# Autodesk Inventor assembly: dxdyrrdtr
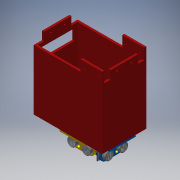
[picture p0: Inventor's stored thumbnail of the model, 180x180]
Saved by Autodesk Inventor 2017 (Build 210142000, 142)
## iProperties
Created: 2017-12-22
Part Number: dxdyrrdtr
Document SubType Name: Assembly
Designer: Dharsan
Author: Dharsan
## Documents named in this file (4)
- C:\Users\Dharsan\Desktop\Dharsan Innovation Files\Cart Model Inventor\Cart Assembly Full.iam
- C:\Users\Dharsan\Desktop\Dharsan Innovation Files\Cart Model Inventor\Cart Body.ipt
- C:\Users\Dharsan\Desktop\Dharsan Innovation Files\Cart Model Inventor\Sensor Hoder and Sensor Assembly.iam
- C:\Users\Dharsan\Desktop\Dharsan Innovation Files\Cart Model Inventor\AS 1427 - M3 x 8(5) II screw.ipt
## Components (7 placed, 3 different names)
1. Cart Body:1 — Mate:8, Mate:9, Mate:10, Mate:11, Mate:12
2. Sensor Hoder and Sensor Assembly:4 [sub-assembly] — Mate:8, Mate:10, Mate:13, Mate:14, Mate:17, Mate:18
3. Sensor Hoder and Sensor Assembly:5 [sub-assembly] — Mate:9, Mate:11, Mate:12, Mate:15, Mate:16, Mate:19, Mate:20
4. AS 1427 - M3 x 8(5) II screw:1 — Mate:19, Mate:20
5. AS 1427 - M3 x 8(5) II screw:2 — Mate:17, Mate:18
6. AS 1427 - M3 x 8(5) II screw:3 — Mate:15, Mate:16
7. AS 1427 - M3 x 8(5) II screw:6 — Mate:13, Mate:14
## Relationships (13: Mate 13)
- Mate:8: Cart Body:1 ↔ Sensor Hoder and Sensor Assembly:4
- Mate:9: Cart Body:1 ↔ Sensor Hoder and Sensor Assembly:5
- Mate:10: Cart Body:1 ↔ Sensor Hoder and Sensor Assembly:4
- Mate:11: Cart Body:1 ↔ Sensor Hoder and Sensor Assembly:5
- Mate:12 (30 mm): Cart Body:1 ↔ Sensor Hoder and Sensor Assembly:5
- Mate:13: Sensor Hoder and Sensor Assembly:4 ↔ AS 1427 - M3 x 8(5) II screw:6
- Mate:14: Sensor Hoder and Sensor Assembly:4 ↔ AS 1427 - M3 x 8(5) II screw:6
- Mate:15: Sensor Hoder and Sensor Assembly:5 ↔ AS 1427 - M3 x 8(5) II screw:3
- Mate:16: Sensor Hoder and Sensor Assembly:5 ↔ AS 1427 - M3 x 8(5) II screw:3
- Mate:17: Sensor Hoder and Sensor Assembly:4 ↔ AS 1427 - M3 x 8(5) II screw:2
- Mate:18: Sensor Hoder and Sensor Assembly:4 ↔ AS 1427 - M3 x 8(5) II screw:2
- Mate:19: Sensor Hoder and Sensor Assembly:5 ↔ AS 1427 - M3 x 8(5) II screw:1
- Mate:20: Sensor Hoder and Sensor Assembly:5 ↔ AS 1427 - M3 x 8(5) II screw:1
